# Autodesk Inventor assembly: ForkMechanism_report
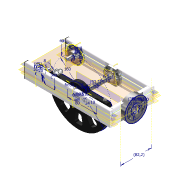
[picture p0: Inventor's stored thumbnail of the model, 180x180]
Saved by Autodesk Inventor 2022 (Build 260153000, 153)
## iProperties
Created: 2022-11-13
Part Number: ForkMechanism_report
Document SubType Name: Assembly
Designer: alexw
Author: alexw
## Documents named in this file (3)
- C:\Users\alexw\Documents\Inventor\Projects\03_CurrentProjects\MasterThesis\PSM_V1_Rillenkugellager\ForkMechanism_report.iam
- C:\Users\alexw\Documents\Inventor\Projects\03_CurrentProjects\MasterThesis\PSM_V1_Rillenkugellager\ParallelMecha_V2_BaseFrame_Item40x40.iam
- C:\Users\alexw\Documents\Inventor\Projects\03_CurrentProjects\MasterThesis\PSM_V1_Rillenkugellager\ContentCenter\de-DE\ISO 4762(2)\ISO 4762 - M5 x 16ISO.ipt
## Components (5 placed, 2 different names)
1. ParallelMecha_V2_BaseFrame_Item40x40:1 [sub-assembly]
2. ISO 4762 M5 x 16:1
3. ISO 4762 M5 x 16:2
4. ISO 4762 M5 x 16:3
5. ISO 4762 M5 x 16:4
## Relationships (8: Mate 8)
- [Mate]: ParallelMecha_V2_BaseFrame_Item40x40:1 ↔ ISO 4762 M5 x 16:1
- [Mate]: ParallelMecha_V2_BaseFrame_Item40x40:1 ↔ ISO 4762 M5 x 16:1
- [Mate]: ParallelMecha_V2_BaseFrame_Item40x40:1 ↔ ISO 4762 M5 x 16:2
- [Mate]: ParallelMecha_V2_BaseFrame_Item40x40:1 ↔ ISO 4762 M5 x 16:2
- [Mate]: ParallelMecha_V2_BaseFrame_Item40x40:1 ↔ ISO 4762 M5 x 16:3
- [Mate]: ParallelMecha_V2_BaseFrame_Item40x40:1 ↔ ISO 4762 M5 x 16:3
- [Mate]: ParallelMecha_V2_BaseFrame_Item40x40:1 ↔ ISO 4762 M5 x 16:4
- [Mate]: ParallelMecha_V2_BaseFrame_Item40x40:1 ↔ ISO 4762 M5 x 16:4
